# Autodesk Inventor assembly: hang arm
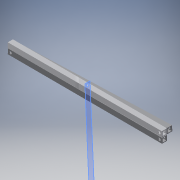
[picture p0: Inventor's stored thumbnail of the model, 180x180]
Saved by Autodesk Inventor 2016 (Build 200138000, 138)
## iProperties
Created: 2016-03-29
Part Number: hang arm
Document SubType Name: Assembly
Designer: gus
Author: gus
## Documents named in this file (6)
- \\Mac\Home\Desktop\1510-stronghold-CAD-master\hang arm 2.0\hang arm.iam
- \\Mac\Home\Desktop\1510-stronghold-CAD-master\hang arm 2.0\support bar.ipt
- \\Mac\Home\Desktop\1510-stronghold-CAD-master\hang arm 2.0\lower arm.ipt
- \\Mac\Home\Desktop\1510-stronghold-CAD-master\hang arm 2.0\upper arm.ipt
- \\Mac\Home\Desktop\1510-stronghold-CAD-master\hang arm 2.0\hool.ipt
- \\Mac\Home\Desktop\1510-stronghold-CAD-master\hang arm 2.0\hook hook.ipt
## Components (5 placed, 5 different names)
1. support bar:1 — Flush:1, Cylindrical:1
2. lower arm:1 — Flush:1, Cylindrical:1, Cylindrical:2, Mate:1
3. upper arm:1 — Cylindrical:2, Mate:1, Flush:2, Cylindrical:3
4. hool:1 — Flush:2, Cylindrical:3, Mate:2, Flush:3, Flush:4
5. hook hook:1 — Mate:2, Flush:3, Flush:4
## Relationships (9: Flush 4, CylindricalJoint 3, Mate 2)
- Flush:1: support bar:1 ↔ lower arm:1
- Cylindrical:1: support bar:1 ↔ lower arm:1
- Cylindrical:2: lower arm:1 ↔ upper arm:1
- Mate:1: lower arm:1 ↔ upper arm:1
- Flush:2: upper arm:1 ↔ hool:1
- Cylindrical:3: upper arm:1 ↔ hool:1
- Mate:2: hool:1 ↔ hook hook:1
- Flush:3: hool:1 ↔ hook hook:1
- Flush:4 (25.4 mm): hool:1 ↔ hook hook:1
